# Autodesk Inventor assembly: UpperBody
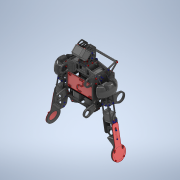
[picture p0: Inventor's stored thumbnail of the model, 180x180]
Saved by Autodesk Inventor 2022 (Build 260153000, 153)
## iProperties
Created: 2022-01-14
Part Number: UpperBody
Document SubType Name: Assembly
Designer: Masato Kubotera
Mass: 1918.95 g
Surface Area: 7006.93 cm^2
Volume: 1229.13 cm^3
Author: Masato Kubotera
## Documents named in this file (9)
- C:\Users\MasatoKubotera\Desktop\SUSTAINA-OP\UpperBody\UpperBody.iam
- C:\Users\MasatoKubotera\Desktop\SUSTAINA-OP\UpperBody\Trunk\Trunk.iam
- C:\Users\MasatoKubotera\Desktop\SUSTAINA-OP\UpperBody\Head\Head.iam
- C:\Users\MasatoKubotera\Desktop\SUSTAINA-OP\UpperBody\Arm\Shoulder.iam
- C:\Users\MasatoKubotera\Desktop\SUSTAINA-OP\UpperBody\Arm\UpperArm.iam
- C:\Users\MasatoKubotera\Desktop\SUSTAINA-OP\UpperBody\Arm\ForeArm.iam
- C:\Users\MasatoKubotera\Desktop\SUSTAINA-OP\UpperBody\Arm\UpperArm_MIR.iam
- C:\Users\MasatoKubotera\Desktop\SUSTAINA-OP\UpperBody\Cockpit\Cockpit.iam
- C:\Users\MasatoKubotera\Desktop\SUSTAINA-OP\UpperBody\Arm\SideBumper.ipt
## Components (11 placed, 8 different names)
1. Trunk:1 [sub-assembly] — フラッシュ:1, フラッシュ:2, フラッシュ:3, 挿入:1, 角度:1, Insert:2, Insert:3, 角度:2, 角度:3, Insert:11
2. Head:1 [sub-assembly] — 挿入:1, 角度:1
3. Shoulder:1 [sub-assembly] — Insert:2, 角度:2, 挿入:4, 角度:4
4. Shoulder:2 [sub-assembly] — Insert:3, 角度:3, Insert:9, Angle:7
5. UpperArm:1 [sub-assembly] — 挿入:4, 角度:4, Insert:6, Angle:6, フラッシュ:4, フラッシュ:5, フラッシュ:6
6. ForeArm:1 [sub-assembly] — Insert:6, Angle:6
7. ForeArm:2 [sub-assembly] — Insert:10, Angle:8
8. UpperArm_MIR:1 [sub-assembly] — Insert:9, Insert:10, Angle:7, Angle:8, メイト:1, メイト:2, フラッシュ:7
9. Cockpit:1 [sub-assembly] — Insert:11, 角度:9
10. SideBumper:1 — フラッシュ:4, フラッシュ:5, フラッシュ:6
11. SideBumper:2 — メイト:1, メイト:2, フラッシュ:7
## Relationships (25: Insert 8, Angle 8, Flush 7, Mate 2)
- フラッシュ:1 [Flush]: Trunk:1
- フラッシュ:2 [Flush]: Trunk:1
- フラッシュ:3 [Flush]: Trunk:1
- 挿入:1 [Insert]: Trunk:1 ↔ Head:1
- 角度:1 [Angle] (180 deg): Trunk:1 ↔ Head:1
- Insert:2: Trunk:1 ↔ Shoulder:1
- Insert:3: Trunk:1 ↔ Shoulder:2
- 角度:2 [Angle] (0 deg): Trunk:1 ↔ Shoulder:1
- 角度:3 [Angle] (0 deg): Trunk:1 ↔ Shoulder:2
- 挿入:4 [Insert]: Shoulder:1 ↔ UpperArm:1
- 角度:4 [Angle] (170 deg): Shoulder:1 ↔ UpperArm:1
- Insert:6: UpperArm:1 ↔ ForeArm:1
- Angle:6 (0 deg): UpperArm:1 ↔ ForeArm:1
- Insert:9: Shoulder:2 ↔ UpperArm_MIR:1
- Insert:10: ForeArm:2 ↔ UpperArm_MIR:1
- Angle:7 (10 deg): Shoulder:2 ↔ UpperArm_MIR:1
- Angle:8 (180 deg): ForeArm:2 ↔ UpperArm_MIR:1
- Insert:11 (0.025 mm): Trunk:1 ↔ Cockpit:1
- 角度:9 [Angle] (0 deg): Cockpit:1
- フラッシュ:4 [Flush]: UpperArm:1 ↔ SideBumper:1
- フラッシュ:5 [Flush]: UpperArm:1 ↔ SideBumper:1
- フラッシュ:6 [Flush]: UpperArm:1 ↔ SideBumper:1
- メイト:1 [Mate]: UpperArm_MIR:1 ↔ SideBumper:2
- メイト:2 [Mate]: UpperArm_MIR:1 ↔ SideBumper:2
- フラッシュ:7 [Flush]: UpperArm_MIR:1 ↔ SideBumper:2
